# Autodesk Inventor assembly: 99455
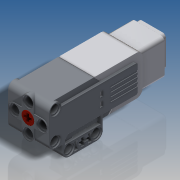
[picture p0: Inventor's stored thumbnail of the model, 180x180]
Saved by Autodesk Inventor 2016 SP2 (Build 200236200, 236)
## iProperties
Created: 2015-09-02
Part Number: 99455
Document SubType Name: Assembly
Designer: D. Kohfeld
Mass: 15.1144 g
Surface Area: 219.045 cm^2
Volume: 14.2589 cm^3
Density: 1.06 g/cm^3
Author: D. Kohfeld
## Documents named in this file (3)
- A:\LEGO Pieces\EV3\99455.iam
- A:\LEGO Pieces\EV3\99535c01.iam
- A:\LEGO Pieces\EV3\99543-Red.ipt
## Components (2 placed, 2 different names)
1. 99535c01:1 [sub-assembly] — Insert:1
2. 99543-Red:1 — Insert:1
## Relationships (1: Insert 1)
- Insert:1: 99535c01:1 ↔ 99543-Red:1
